# Autodesk Inventor assembly: USB_Board_asy
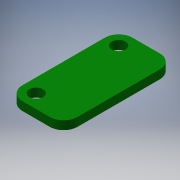
[picture p0: Inventor's stored thumbnail of the model, 180x180]
Saved by Autodesk Inventor 2017 (Build 210142000, 142)
## iProperties
Created: 2017-08-03
Part Number: USB_Board_asy
Document SubType Name: Assembly
Designer: Mitch
Author: Mitch
## Documents named in this file (3)
- E:\Youtube Channel\Pojects\Brew Probe\USB_Board_asy.iam
- E:\Youtube Channel\Pojects\Brew Probe\USB_Board.ipt
- E:\Youtube Channel\Pojects\Brew Probe\micro usb.ipt
## Components (2 placed, 2 different names)
1. USB_Board:1 — Mate:1, Flush:1, Mate:2
2. micro usb:1 — Mate:1, Flush:1, Mate:3
## Relationships (5: Mate 3, Flush 2)
- Mate:1: USB_Board:1 ↔ micro usb:1
- Flush:1: USB_Board:1 ↔ micro usb:1
- Mate:2: USB_Board:1
- Flush:2 (6.35 mm)
- Mate:3: micro usb:1
